# Autodesk Inventor assembly: Impulsor
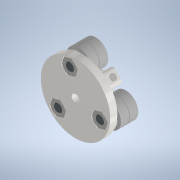
[picture p0: Inventor's stored thumbnail of the model, 180x180]
Saved by Autodesk Inventor 2020.2 (Build 242310000, 310)
## iProperties
Created: 2020-09-07
Part Number: Impulsor
Document SubType Name: Assembly
Designer: JK
Author: JK
## Documents named in this file (7)
- C:\Users\JK\Documents\Inventor\BioMixer\BombaPeristaltica\Impulsor.iam
- C:\Users\JK\Documents\Inventor\BioMixer\BombaPeristaltica\Impulsor.ipt
- C:\Users\JK\Documents\Inventor\BioMixer\BombaPeristaltica\TuercaM5BajoPerfil.ipt
- C:\Users\JK\Documents\Inventor\BioMixer\BombaPeristaltica\PrisioneroM3x6.ipt
- C:\Users\JK\Documents\Inventor\BioMixer\BombaPeristaltica\TuercaM3.ipt
- C:\Users\JK\Documents\Inventor\BioMixer\BombaPeristaltica\PernoM5x15Plano.ipt
- C:\Users\JK\Documents\Inventor\BioMixer\BombaPeristaltica\605ZZ\Rodamiento605ZZ.iam
## Components (19 placed, 6 different names)
1. Impulsor — Flush:5, Angle:1, Angle:2, Angle:3, Mate:19, Mate:20, Mate:21, Angle:4, Angle:5, Angle:6, Mate:22, Mate:23, Mate:24, Mate:25, Mate:26, Mate:27, Flush:6, Flush:7, Flush:8, Mate:34, Mate:35, Mate:36, Mate:37
2. PernoM5x15Plano:1 — Flush:3, Mate:38, Mate:39
3. PernoM5x15Plano:2 — Flush:3, Flush:4
4. PernoM5x15Plano:3 — Flush:4, Mate:18
5. TuercaM5BajoPerfil:1 — Flush:2, Mate:18, Flush:5, Angle:1
6. TuercaM5BajoPerfil:2 — Flush:1, Flush:2, Angle:3
7. TuercaM5BajoPerfil:3 — Flush:1, Angle:2
8. TuercaM3:1 — Mate:21, Angle:6, Mate:23
9. TuercaM3:2 — Mate:20, Angle:5, Mate:24
10. TuercaM3:3 — Mate:19, Angle:4, Mate:22
11. PrisioneroM3x6:1 — Mate:25, Flush:6
12. PrisioneroM3x6:2 — Mate:26, Flush:7
13. PrisioneroM3x6:3 — Mate:27, Flush:8
14. Rodamiento605ZZ:1 [sub-assembly] — Mate:28, Mate:29, Mate:37
15. Rodamiento605ZZ:2 [sub-assembly] — Mate:28, Mate:29, Mate:34, Flush:9, Flush:10
16. Rodamiento605ZZ:3 [sub-assembly] — Mate:30, Mate:32, Mate:35, Flush:10, Mate:38, Mate:39
17. Rodamiento605ZZ:4 [sub-assembly] — Mate:30, Mate:32
18. Rodamiento605ZZ:5 [sub-assembly] — Mate:31, Mate:33, Mate:36, Flush:9
19. Rodamiento605ZZ:6 [sub-assembly] — Mate:31, Mate:33
## Relationships (38: Mate 22, Flush 10, Angle 6)
- Flush:1: TuercaM5BajoPerfil:2 ↔ TuercaM5BajoPerfil:3
- Flush:2: TuercaM5BajoPerfil:1 ↔ TuercaM5BajoPerfil:2
- Flush:3: PernoM5x15Plano:1 ↔ PernoM5x15Plano:2
- Flush:4: PernoM5x15Plano:2 ↔ PernoM5x15Plano:3
- Mate:18: PernoM5x15Plano:3 ↔ TuercaM5BajoPerfil:1
- Flush:5: Impulsor ↔ TuercaM5BajoPerfil:1
- Angle:1 (0 deg): Impulsor ↔ TuercaM5BajoPerfil:1
- Angle:2 (0 deg): Impulsor ↔ TuercaM5BajoPerfil:3
- Angle:3 (0 deg): Impulsor ↔ TuercaM5BajoPerfil:2
- Mate:19: Impulsor ↔ TuercaM3:3
- Mate:20: Impulsor ↔ TuercaM3:2
- Mate:21: Impulsor ↔ TuercaM3:1
- Angle:4 (0 deg): Impulsor ↔ TuercaM3:3
- Angle:5 (0 deg): Impulsor ↔ TuercaM3:2
- Angle:6 (0 deg): Impulsor ↔ TuercaM3:1
- Mate:22: Impulsor ↔ TuercaM3:3
- Mate:23: Impulsor ↔ TuercaM3:1
- Mate:24: Impulsor ↔ TuercaM3:2
- Mate:25: Impulsor ↔ PrisioneroM3x6:1
- Mate:26: Impulsor ↔ PrisioneroM3x6:2
- Mate:27: Impulsor ↔ PrisioneroM3x6:3
- Flush:6 (4 mm): Impulsor ↔ PrisioneroM3x6:1
- Flush:7 (4 mm): Impulsor ↔ PrisioneroM3x6:2
- Flush:8 (4 mm): Impulsor ↔ PrisioneroM3x6:3
- Mate:28: Rodamiento605ZZ:1 ↔ Rodamiento605ZZ:2
- Mate:29: Rodamiento605ZZ:1 ↔ Rodamiento605ZZ:2
- Mate:30: Rodamiento605ZZ:3 ↔ Rodamiento605ZZ:4
- Mate:31: Rodamiento605ZZ:5 ↔ Rodamiento605ZZ:6
- Mate:32: Rodamiento605ZZ:3 ↔ Rodamiento605ZZ:4
- Mate:33: Rodamiento605ZZ:5 ↔ Rodamiento605ZZ:6
- Mate:34: Impulsor ↔ Rodamiento605ZZ:2
- Mate:35: Impulsor ↔ Rodamiento605ZZ:3
- Mate:36: Impulsor ↔ Rodamiento605ZZ:5
- Flush:9: Rodamiento605ZZ:2 ↔ Rodamiento605ZZ:5
- Flush:10: Rodamiento605ZZ:2 ↔ Rodamiento605ZZ:3
- Mate:37: Impulsor ↔ Rodamiento605ZZ:1
- Mate:38: PernoM5x15Plano:1 ↔ Rodamiento605ZZ:3
- Mate:39: PernoM5x15Plano:1 ↔ Rodamiento605ZZ:3
